# Autodesk Inventor assembly: SG90 - Micro Servo 9g - Tower Pro
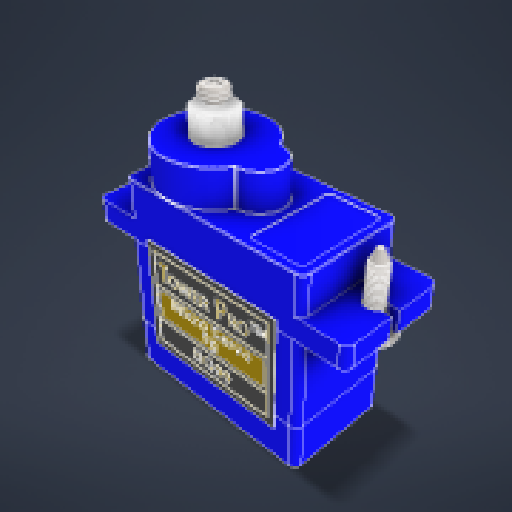
[picture p0: Inventor's stored thumbnail of the model, 512x512]
Saved by Autodesk Inventor 2025 (Build 290162000, 162)
## iProperties
Created: 2024-05-24
Part Number: SG90 - Micro Servo 9g - Tower Pro
Document SubType Name: Assembly
Designer: Garfieldcmix
Sending System: SOLIDWORKS 2016-2016095
MC: AMD64
MC_MODEL: Intel64 Family 6 Model 142 Stepping 9, GenuineIntel
OS: Windows_NT
FRU: Parasolid Version 28.0, build 209,  1-25-2016
FORMAT: text
GUISE: transmit
KEY: SG90 - Micro Servo 9g - Tower Pro
FILE: SG90 - Micro Servo 9g - Tower Pro.x_t
DATE: Sat Nov 11 17:21:38 2017
Author: Garfieldcmix
## Documents named in this file (16)
- C:\Users\chaya\Desktop\WRO-2024-CAD\SG90 - Micro Servo 9g - Tower Pro\SG90 - Micro Servo 9g - Tower Pro.iam
- C:\Users\chaya\Desktop\WRO-2024-CAD\SG90 - Micro Servo 9g - Tower Pro\Tower Pro - Micro Servo 9g - SG90.1.ipt
- C:\Users\chaya\Desktop\WRO-2024-CAD\SG90 - Micro Servo 9g - Tower Pro\Tower Pro - Micro Servo 9g - SG90.1_1.ipt
- C:\Users\chaya\Desktop\WRO-2024-CAD\SG90 - Micro Servo 9g - Tower Pro\Tower Pro - Micro Servo 9g - SG90.1_2.ipt
- C:\Users\chaya\Desktop\WRO-2024-CAD\SG90 - Micro Servo 9g - Tower Pro\Tower Pro - Micro Servo 9g - SG90.1_3.ipt
- C:\Users\chaya\Desktop\WRO-2024-CAD\SG90 - Micro Servo 9g - Tower Pro\Tower Pro - Micro Servo 9g - SG90.1_4.ipt
- C:\Users\chaya\Desktop\WRO-2024-CAD\SG90 - Micro Servo 9g - Tower Pro\Tower Pro - Micro Servo 9g - SG90.1_5.ipt
- C:\Users\chaya\Desktop\WRO-2024-CAD\SG90 - Micro Servo 9g - Tower Pro\Tower Pro - Micro Servo 9g - SG90.1_6.ipt
- C:\Users\chaya\Desktop\WRO-2024-CAD\SG90 - Micro Servo 9g - Tower Pro\Tower Pro - Micro Servo 9g - SG90.1_7.ipt
- C:\Users\chaya\Desktop\WRO-2024-CAD\SG90 - Micro Servo 9g - Tower Pro\Tower Pro - Micro Servo 9g - SG90.1_8.ipt
- C:\Users\chaya\Desktop\WRO-2024-CAD\SG90 - Micro Servo 9g - Tower Pro\Tower Pro - Micro Servo 9g - SG90.1_9.ipt
- C:\Users\chaya\Desktop\WRO-2024-CAD\SG90 - Micro Servo 9g - Tower Pro\Tower Pro - Micro Servo 9g - SG90.1_10.ipt
- C:\Users\chaya\Desktop\WRO-2024-CAD\SG90 - Micro Servo 9g - Tower Pro\Tower Pro - Micro Servo 9g - SG90.1_11.ipt
- C:\Users\chaya\Desktop\WRO-2024-CAD\SG90 - Micro Servo 9g - Tower Pro\Tower Pro - Micro Servo 9g - SG90.1_12.ipt
- C:\Users\chaya\Desktop\WRO-2024-CAD\SG90 - Micro Servo 9g - Tower Pro\SG90 - Micro Servo 9g - Tower Pro.5.ipt
- C:\Users\chaya\Desktop\WRO-2024-CAD\SG90 - Micro Servo 9g - Tower Pro\SG90 - Micro Servo 9g - Tower Pro.6.ipt
## Components (16 placed, 15 different names)
1. Tower Pro - Micro Servo 9g - SG90.1
2. Tower Pro - Micro Servo 9g - SG90.1_1
3. Tower Pro - Micro Servo 9g - SG90.1_2
4. Tower Pro - Micro Servo 9g - SG90.1_3
5. Tower Pro - Micro Servo 9g - SG90.1_4
6. Tower Pro - Micro Servo 9g - SG90.1_5
7. Tower Pro - Micro Servo 9g - SG90.1_6
8. Tower Pro - Micro Servo 9g - SG90.1_7
9. Tower Pro - Micro Servo 9g - SG90.1_8
10. Tower Pro - Micro Servo 9g - SG90.1_9
11. Tower Pro - Micro Servo 9g - SG90.1_10
12. Tower Pro - Micro Servo 9g - SG90.1_11 — Mate:1, Mate:2, Mate:3, Mate:4
13. Tower Pro - Micro Servo 9g - SG90.1_12
14. SG90 - Micro Servo 9g - Tower Pro.5 — Mate:3, Mate:4
15. SG90 - Micro Servo 9g - Tower Pro.5:1 — Mate:1, Mate:2
16. SG90 - Micro Servo 9g - Tower Pro.6
## Relationships (4: Mate 4)
- Mate:1: Tower Pro - Micro Servo 9g - SG90.1_11 ↔ SG90 - Micro Servo 9g - Tower Pro.5:1
- Mate:2: Tower Pro - Micro Servo 9g - SG90.1_11 ↔ SG90 - Micro Servo 9g - Tower Pro.5:1
- Mate:3: Tower Pro - Micro Servo 9g - SG90.1_11 ↔ SG90 - Micro Servo 9g - Tower Pro.5
- Mate:4: Tower Pro - Micro Servo 9g - SG90.1_11 ↔ SG90 - Micro Servo 9g - Tower Pro.5
